# Autodesk Inventor assembly: Assembly_Cube_AlliedVision_Alvium_Bareboard
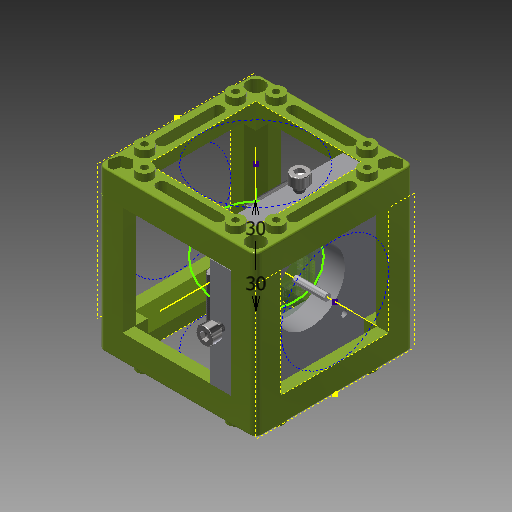
[picture p0: Inventor's stored thumbnail of the model, 512x512]
Saved by Autodesk Inventor 2019 (Build 230136000, 136)
## iProperties
Created: 2019-07-24
Part Number: Assembly_Cube_AlliedVision_Alvium_Bareboard
Document SubType Name: Assembly
Designer: marsikovabarbora
Mass: 80.2246 g
Surface Area: 390.041 cm^2
Volume: 68.7061 cm^3
Density: 1.16765 g/cm^3
Author: marsikovabarbora
## Documents named in this file (5)
- C:\Users\marsikovabarbora\Dropbox\UC2\02_CAD\INVENTOR\uc2_v3\Assembly_Cube_AlliedVision_Alvium_Bareboard.iam
- C:\Users\marsikovabarbora\Dropbox\UC2\02_CAD\INVENTOR\uc2_v3\Assembly_Cube_empty_IM_v3.iam
- C:\Users\marsikovabarbora\Documents\Inventor\Content Center Files\R2019\en-US\DIN 912\DIN 912 - M3 x 0,5 x 16 x 14,75.ipt
- C:\Users\marsikovabarbora\Dropbox\UC2\02_CAD\INVENTOR\uc2_v3\20_Cube_Insert_AlliedVision_Alvium_Bareboard_v3.ipt
- C:\Users\marsikovabarbora\Dropbox\UC2\02_CAD\INVENTOR\uc2_v3\00_Alvium_Step_USB180_CS-Mount_OpenHousing_2019-Mar-28.ipt
## Components (7 placed, 4 different names)
1. Assembly_Cube_empty_IM_v3:1 [sub-assembly] — Mate:1, Mate:2, Mate:3, Mate:4, Mate:16, Mate:18, Angle:2
2. 20_Cube_Insert_AlliedVision_Alvium_Bareboard_v3:1 — Mate:12, Mate:14, Mate:16, Mate:18, Angle:2, Mate:19, Flush:3, Flush:4, Mate:20, Angle:3, Mate:21
3. DIN 912 - replaced by DIN EN ISO 4762 M3 x 16:1 — Mate:19, Flush:4
4. DIN 912 - replaced by DIN EN ISO 4762 M3 x 16:2 — Mate:12
5. DIN 912 - replaced by DIN EN ISO 4762 M3 x 16:3
6. DIN 912 - replaced by DIN EN ISO 4762 M3 x 16:4 — Mate:14, Flush:3
7. 00_Alvium_Step_USB180_CS-Mount_OpenHousing_2019-Mar-28:1 — Mate:20, Angle:3, Mate:21
## Relationships (15: Mate 11, Angle 2, Flush 2)
- Mate:1: Assembly_Cube_empty_IM_v3:1
- Mate:2: Assembly_Cube_empty_IM_v3:1
- Mate:3: Assembly_Cube_empty_IM_v3:1
- Mate:4: Assembly_Cube_empty_IM_v3:1
- Mate:12: 20_Cube_Insert_AlliedVision_Alvium_Bareboard_v3:1 ↔ DIN 912 - replaced by DIN EN ISO 4762 M3 x 16:2
- Mate:14: 20_Cube_Insert_AlliedVision_Alvium_Bareboard_v3:1 ↔ DIN 912 - replaced by DIN EN ISO 4762 M3 x 16:4
- Mate:16: Assembly_Cube_empty_IM_v3:1 ↔ 20_Cube_Insert_AlliedVision_Alvium_Bareboard_v3:1
- Mate:18: Assembly_Cube_empty_IM_v3:1 ↔ 20_Cube_Insert_AlliedVision_Alvium_Bareboard_v3:1
- Angle:2 (0 deg): Assembly_Cube_empty_IM_v3:1 ↔ 20_Cube_Insert_AlliedVision_Alvium_Bareboard_v3:1
- Mate:19: 20_Cube_Insert_AlliedVision_Alvium_Bareboard_v3:1 ↔ DIN 912 - replaced by DIN EN ISO 4762 M3 x 16:1
- Flush:3 (-5 mm): 20_Cube_Insert_AlliedVision_Alvium_Bareboard_v3:1 ↔ DIN 912 - replaced by DIN EN ISO 4762 M3 x 16:4
- Flush:4 (5 mm): 20_Cube_Insert_AlliedVision_Alvium_Bareboard_v3:1 ↔ DIN 912 - replaced by DIN EN ISO 4762 M3 x 16:1
- Mate:20: 20_Cube_Insert_AlliedVision_Alvium_Bareboard_v3:1 ↔ 00_Alvium_Step_USB180_CS-Mount_OpenHousing_2019-Mar-28:1
- Angle:3 (180 deg): 20_Cube_Insert_AlliedVision_Alvium_Bareboard_v3:1 ↔ 00_Alvium_Step_USB180_CS-Mount_OpenHousing_2019-Mar-28:1
- Mate:21: 20_Cube_Insert_AlliedVision_Alvium_Bareboard_v3:1 ↔ 00_Alvium_Step_USB180_CS-Mount_OpenHousing_2019-Mar-28:1
